# Autodesk Inventor assembly: Marco_Conveyor_Aereo
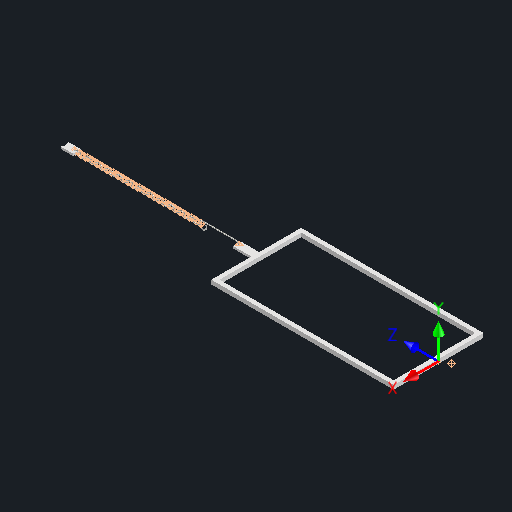
[picture p0: Inventor's stored thumbnail of the model, 512x512]
Saved by Autodesk Inventor 2024 (Build 280153000, 153)
## iProperties
Created: 2023-05-13
Part Number: Marco_Conveyor_Aereo
Document SubType Name: Assembly
Designer: javie
Author: javie
## Documents named in this file (4)
- C:\Users\javie\Downloads\Piezas CMR\Marco_Conveyor_Aereo.iam
- C:\Users\javie\Downloads\cadena-chain-2.snapshot.2\cadena.ipt
- C:\Users\javie\Downloads\cadena-chain-2.snapshot.2\Gancho.ipt
- C:\Users\javie\Downloads\cadena-chain-2.snapshot.2\Marco.ipt
## Components (26 placed, 3 different names)
1. cadena:1 — Coincidencia:1, Coincidencia:2
2. cadena:2 — Coincidencia:1, Coincidencia:3
3. cadena:3 — Coincidencia:4, Coincidencia:5
4. cadena:4 — Coincidencia:3, Coincidencia:26, Coincidencia:27
5. cadena:5 — Coincidencia:2, Coincidencia:4
6. cadena:6 — Coincidencia:5, Coincidencia:11
7. cadena:7
8. cadena:8
9. cadena:9
10. cadena:10 — Coincidencia:11
11. cadena:11
12. cadena:12 — Coincidencia:23
13. cadena:13
14. cadena:14
15. cadena:15
16. cadena:16 — Coincidencia:23
17. cadena:17
18. cadena:18
19. cadena:19
20. cadena:20
21. cadena:21
22. cadena:22
23. cadena:23
24. cadena:24 — Coincidencia:24, Coincidencia:25
25. Gancho:1 — Coincidencia:24, Coincidencia:25
26. Marco:1 — Coincidencia:26, Coincidencia:27
## Relationships (27: Mate 27)
- Coincidencia:1 [Mate]: cadena:1 ↔ cadena:2
- Coincidencia:2 [Mate]: cadena:1 ↔ cadena:5
- Coincidencia:3 [Mate]: cadena:2 ↔ cadena:4
- Coincidencia:4 [Mate]: cadena:3 ↔ cadena:5
- Coincidencia:5 [Mate]: cadena:3 ↔ cadena:6
- [Mate]: cadena:7 ↔ cadena:8
- [Mate]: cadena:7 ↔ cadena:11
- [Mate]: cadena:8 ↔ cadena:10
- [Mate]: cadena:9 ↔ cadena:11
- [Mate]: cadena:9 ↔ cadena:12
- Coincidencia:11 [Mate]: cadena:6 ↔ cadena:10
- [Mate]: cadena:13 ↔ cadena:14
- [Mate]: cadena:13 ↔ cadena:17
- [Mate]: cadena:14 ↔ cadena:16
- [Mate]: cadena:15 ↔ cadena:17
- [Mate]: cadena:15 ↔ cadena:18
- [Mate]: cadena:19 ↔ cadena:20
- [Mate]: cadena:19 ↔ cadena:23
- [Mate]: cadena:20 ↔ cadena:22
- [Mate]: cadena:21 ↔ cadena:23
- [Mate]: cadena:21 ↔ cadena:24
- [Mate]: cadena:18 ↔ cadena:22
- Coincidencia:23 [Mate]: cadena:12 ↔ cadena:16
- Coincidencia:24 [Mate]: cadena:24 ↔ Gancho:1
- Coincidencia:25 [Mate]: cadena:24 ↔ Gancho:1
- Coincidencia:26 [Mate]: cadena:4 ↔ Marco:1
- Coincidencia:27 [Mate]: cadena:4 ↔ Marco:1
## Named parameters: d6_d2 = 0 mm, d7_d3 = 0 mm, d8_d4 = 0 mm, d9_d5 = 0 mm, d10_d1 = 0 mm, d12_d2 = 0 mm, d13_d3 = 0 mm, d14_d4 = 0 mm, d15_d5 = 0 mm, d16_d6_d2 = 0 mm, d17_d7_d3 = 0 mm, d18_d8_d4 = 0 mm, d19_d9_d5 = 0 mm, d20_d10_d1 = 0 mm, d21_d11 = 0 mm, d22_d1 = 0 mm
